# Autodesk Inventor assembly: wheel
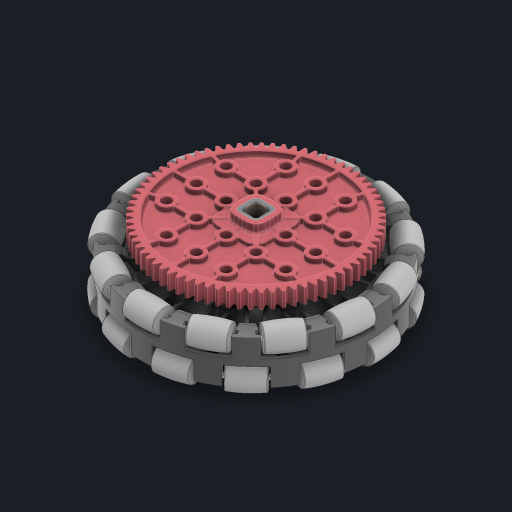
[picture p0: Inventor's stored thumbnail of the model, 512x512]
Saved by Autodesk Inventor 2024 (Build 280153000, 153)
## iProperties
Created: 2023-08-15
Part Number: wheel
Document SubType Name: Assembly
Designer: avere
Author: avere
## Documents named in this file (4)
- D:\vex_robotics\hardware\cad\scrap_v0.1\chassis\wheel.iam
- D:\vex_robotics\hardware\cad\VEX-CAD-Inventor-1.41\Motion\Wheels\Omni Wheel\4 Omni AS, No Insert.iam
- D:\vex_robotics\hardware\cad\scrap_v0.1\chassis\custom_parts\half_cut_72.ipt
- D:\vex_robotics\hardware\cad\VEX-CAD-Inventor-1.41\Motion\Wheels\Omni Wheel.iam
## Components (2 placed, 2 different names)
1. half_cut_72:1 — Insert:1, Mate:1
2. 4 Omni AS, No Insert:1 [sub-assembly] — Insert:1, Mate:1
## Relationships (2: Insert 1, Mate 1)
- Insert:1 (3.175 mm): half_cut_72:1 ↔ 4 Omni AS, No Insert:1
- Mate:1: half_cut_72:1 ↔ 4 Omni AS, No Insert:1
